# Autodesk Inventor assembly: new collector mount
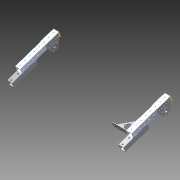
[picture p0: Inventor's stored thumbnail of the model, 180x180]
Saved by Autodesk Inventor 2014 SP1 (Build 180222100, 222)
## iProperties
Created: 2014-01-17
Part Number: new collector mount
Document SubType Name: Assembly
Designer: Arpan
Author: Arpan
## Documents named in this file (6)
- C:\Users\Arpan\Documents\GitHub\2014buildCAD\new collector mount\new collector mount.iam
- C:\Users\Arpan\Documents\GitHub\2014buildCAD\new collector mount\Vex Pro 1x1 rectangular tubing 9 in length.ipt
- C:\Users\Arpan\Documents\GitHub\2014buildCAD\new collector mount\Vex Pro Side Bearing Gusset.ipt
- C:\Users\Arpan\Documents\GitHub\2014buildCAD\new collector mount\Vex Pro Corner Gusset.ipt
- C:\Users\Arpan\Documents\GitHub\2014buildCAD\New Collector\Hex Bearing 1-2 in (FR8ZZ-Hex, am-0279).ipt
- C:\Users\Arpan\Documents\GitHub\2014buildCAD\new collector mount\Square Tube 1-16 thick Support.ipt
## Components (13 placed, 5 different names)
1. Vex Pro 1x1 rectangular tubing 9 in length:1 — Mate:1, Flush:1, Flush:2, Mate:10, Mate:13, Mate:17, Mate:18, Mate:19, Mate:40, Mate:41, Mate:42, Mate:43, Mate:48, Mate:65, Mate:66
2. Vex Pro 1x1 rectangular tubing 9 in length:2 — Mate:1, Flush:1, Flush:2, Mate:4, Mate:7, Mate:36, Mate:37, Mate:38, Mate:39, Mate:45, Mate:46, Mate:47
3. Vex Pro Side Bearing Gusset:1 — Mate:4, Mate:24, Mate:25, Mate:38, Mate:39
4. Vex Pro Side Bearing Gusset:2 — Mate:7, Mate:26, Mate:27, Mate:36, Mate:37
5. Vex Pro Side Bearing Gusset:3 — Mate:10, Mate:20, Mate:21, Mate:42, Mate:43
6. Vex Pro Side Bearing Gusset:4 — Mate:13, Mate:22, Mate:23, Mate:40, Mate:41
7. Vex Pro Corner Gusset:2 — Mate:17, Mate:18, Mate:19
8. Hex Bearing 1-2 in (FR8ZZ-Hex, am-0279):1 — Mate:20, Mate:21, Flush:4, Flush:5
9. Hex Bearing 1-2 in (FR8ZZ-Hex, am-0279):2 — Mate:22, Mate:23, Flush:4
10. Hex Bearing 1-2 in (FR8ZZ-Hex, am-0279):3 — Mate:24, Mate:25, Flush:3
11. Hex Bearing 1-2 in (FR8ZZ-Hex, am-0279):4 — Mate:26, Mate:27, Flush:3, Flush:5
12. Square Tube 1-16 thick Support:1 — Mate:45, Mate:46, Mate:47
13. Square Tube 1-16 thick Support:2 — Mate:48, Mate:65, Mate:66
## Relationships (35: Mate 30, Flush 5)
- Mate:1 (533.4 mm): Vex Pro 1x1 rectangular tubing 9 in length:1 ↔ Vex Pro 1x1 rectangular tubing 9 in length:2
- Flush:1: Vex Pro 1x1 rectangular tubing 9 in length:1 ↔ Vex Pro 1x1 rectangular tubing 9 in length:2
- Flush:2: Vex Pro 1x1 rectangular tubing 9 in length:1 ↔ Vex Pro 1x1 rectangular tubing 9 in length:2
- Mate:4: Vex Pro 1x1 rectangular tubing 9 in length:2 ↔ Vex Pro Side Bearing Gusset:1
- Mate:7: Vex Pro 1x1 rectangular tubing 9 in length:2 ↔ Vex Pro Side Bearing Gusset:2
- Mate:10: Vex Pro 1x1 rectangular tubing 9 in length:1 ↔ Vex Pro Side Bearing Gusset:3
- Mate:13: Vex Pro 1x1 rectangular tubing 9 in length:1 ↔ Vex Pro Side Bearing Gusset:4
- Mate:17: Vex Pro 1x1 rectangular tubing 9 in length:1 ↔ Vex Pro Corner Gusset:2
- Mate:18: Vex Pro 1x1 rectangular tubing 9 in length:1 ↔ Vex Pro Corner Gusset:2
- Mate:19: Vex Pro 1x1 rectangular tubing 9 in length:1 ↔ Vex Pro Corner Gusset:2
- Mate:20: Vex Pro Side Bearing Gusset:3 ↔ Hex Bearing 1-2 in (FR8ZZ-Hex, am-0279):1
- Mate:21: Vex Pro Side Bearing Gusset:3 ↔ Hex Bearing 1-2 in (FR8ZZ-Hex, am-0279):1
- Mate:22: Vex Pro Side Bearing Gusset:4 ↔ Hex Bearing 1-2 in (FR8ZZ-Hex, am-0279):2
- Mate:23: Vex Pro Side Bearing Gusset:4 ↔ Hex Bearing 1-2 in (FR8ZZ-Hex, am-0279):2
- Mate:24: Vex Pro Side Bearing Gusset:1 ↔ Hex Bearing 1-2 in (FR8ZZ-Hex, am-0279):3
- Mate:25: Vex Pro Side Bearing Gusset:1 ↔ Hex Bearing 1-2 in (FR8ZZ-Hex, am-0279):3
- Mate:26: Vex Pro Side Bearing Gusset:2 ↔ Hex Bearing 1-2 in (FR8ZZ-Hex, am-0279):4
- Mate:27: Vex Pro Side Bearing Gusset:2 ↔ Hex Bearing 1-2 in (FR8ZZ-Hex, am-0279):4
- Flush:3: Hex Bearing 1-2 in (FR8ZZ-Hex, am-0279):3 ↔ Hex Bearing 1-2 in (FR8ZZ-Hex, am-0279):4
- Flush:4: Hex Bearing 1-2 in (FR8ZZ-Hex, am-0279):1 ↔ Hex Bearing 1-2 in (FR8ZZ-Hex, am-0279):2
- Flush:5: Hex Bearing 1-2 in (FR8ZZ-Hex, am-0279):1 ↔ Hex Bearing 1-2 in (FR8ZZ-Hex, am-0279):4
- Mate:36: Vex Pro 1x1 rectangular tubing 9 in length:2 ↔ Vex Pro Side Bearing Gusset:2
- Mate:37: Vex Pro 1x1 rectangular tubing 9 in length:2 ↔ Vex Pro Side Bearing Gusset:2
- Mate:38: Vex Pro 1x1 rectangular tubing 9 in length:2 ↔ Vex Pro Side Bearing Gusset:1
- Mate:39: Vex Pro 1x1 rectangular tubing 9 in length:2 ↔ Vex Pro Side Bearing Gusset:1
- Mate:40: Vex Pro 1x1 rectangular tubing 9 in length:1 ↔ Vex Pro Side Bearing Gusset:4
- Mate:41: Vex Pro 1x1 rectangular tubing 9 in length:1 ↔ Vex Pro Side Bearing Gusset:4
- Mate:42: Vex Pro 1x1 rectangular tubing 9 in length:1 ↔ Vex Pro Side Bearing Gusset:3
- Mate:43: Vex Pro 1x1 rectangular tubing 9 in length:1 ↔ Vex Pro Side Bearing Gusset:3
- Mate:45: Vex Pro 1x1 rectangular tubing 9 in length:2 ↔ Square Tube 1-16 thick Support:1
- Mate:46: Vex Pro 1x1 rectangular tubing 9 in length:2 ↔ Square Tube 1-16 thick Support:1
- Mate:47: Vex Pro 1x1 rectangular tubing 9 in length:2 ↔ Square Tube 1-16 thick Support:1
- Mate:48: Vex Pro 1x1 rectangular tubing 9 in length:1 ↔ Square Tube 1-16 thick Support:2
- Mate:65: Vex Pro 1x1 rectangular tubing 9 in length:1 ↔ Square Tube 1-16 thick Support:2
- Mate:66: Vex Pro 1x1 rectangular tubing 9 in length:1 ↔ Square Tube 1-16 thick Support:2
